# Autodesk Inventor assembly: Base
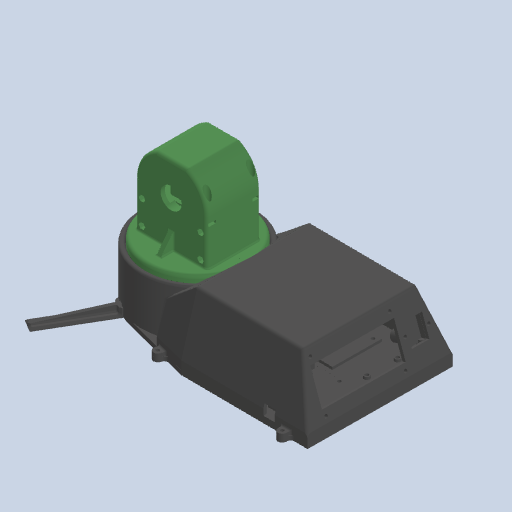
[picture p0: Inventor's stored thumbnail of the model, 512x512]
Saved by Autodesk Inventor 2023 (Build 270158000, 158)
## iProperties
Created: 2024-07-31
Part Number: Base
Document SubType Name: Assembly
Designer: Swoby
Author: Swoby
## Documents named in this file (10)
- C:\Users\Swoby\OneDrive\Plocha\DUM-E\V0.3\NewBase\Base.iam
- C:\Users\Swoby\OneDrive\Plocha\DUM-E\V0.3\NewBase\Base_1L.ipt
- C:\Users\Swoby\OneDrive\Plocha\DUM-E\V0.3\NewBase\Base_1R.ipt
- C:\Users\Swoby\OneDrive\Plocha\DUM-E\V0.3\NewBase\Base_1Up.ipt
- C:\Users\Swoby\OneDrive\Plocha\DUM-E\V0.3\NewBase\Base_2R.ipt
- C:\Users\Swoby\OneDrive\Plocha\DUM-E\V0.3\NewBase\Base_2Leg.ipt
- C:\Users\Swoby\OneDrive\Plocha\DUM-E\V0.3\NewBase\Base_2L.ipt
- C:\Users\Swoby\OneDrive\Plocha\DUM-E\V0.3\NewBase\Clamp_Holder.ipt
- C:\Users\Swoby\OneDrive\Plocha\DUM-E\V0.3\NewBase\Base_Cover.ipt
- C:\Users\Swoby\OneDrive\Plocha\DUM-E\V0.3\NewBase\KeyPad_Holder.ipt
## Components (11 placed, 9 different names)
1. Base_1L:1 — Mate:1, Mate:2, Mate:3, Mate:5, Mate:6, Mate:7, Mate:8
2. Base_1R:1 — Mate:1, Mate:2, Mate:3, Mate:4
3. Base_1Up:1 — Mate:4, Mate:5, Mate:6
4. Base_2R:1 — Mate:7, Mate:8, Mate:11, Mate:12, Mate:13, Flush:3, Mate:16, Mate:17
5. Base_2Leg:1 — Flush:3, Mate:16, Mate:17
6. Base_2L:1 — Mate:11, Mate:12, Mate:13, Mate:14, Flush:2, Mate:15, Mate:18, Mate:19, Mate:20, Mate:21, Mate:22, Mate:23, Flush:4, Flush:5, Mate:24
7. Base_2Leg:2 — Mate:14, Flush:2, Mate:15
8. Clamp_Holder:1 — Mate:18, Mate:19, Mate:22
9. Clamp_Holder:2 — Mate:20, Mate:21, Mate:23
10. Base_Cover:1 — Flush:4, Flush:5, Mate:24, Mate:25, Mate:26, Mate:27
11. KeyPad_Holder:1 — Mate:25, Mate:26, Mate:27
## Relationships (29: Mate 25, Flush 4)
- Mate:1: Base_1L:1 ↔ Base_1R:1
- Mate:2: Base_1L:1 ↔ Base_1R:1
- Mate:3: Base_1L:1 ↔ Base_1R:1
- Mate:4: Base_1R:1 ↔ Base_1Up:1
- Mate:5: Base_1L:1 ↔ Base_1Up:1
- Mate:6: Base_1L:1 ↔ Base_1Up:1
- Mate:7 (0.5 mm): Base_1L:1 ↔ Base_2R:1
- Mate:8: Base_1L:1 ↔ Base_2R:1
- Mate:11: Base_2R:1 ↔ Base_2L:1
- Mate:12: Base_2R:1 ↔ Base_2L:1
- Mate:13: Base_2R:1 ↔ Base_2L:1
- Mate:14: Base_2L:1 ↔ Base_2Leg:2
- Flush:2: Base_2L:1 ↔ Base_2Leg:2
- Mate:15 (0.3 mm): Base_2L:1 ↔ Base_2Leg:2
- Flush:3: Base_2R:1 ↔ Base_2Leg:1
- Mate:16: Base_2R:1 ↔ Base_2Leg:1
- Mate:17 (0.3 mm): Base_2R:1 ↔ Base_2Leg:1
- Mate:18: Base_2L:1 ↔ Clamp_Holder:1
- Mate:19: Base_2L:1 ↔ Clamp_Holder:1
- Mate:20: Base_2L:1 ↔ Clamp_Holder:2
- Mate:21: Base_2L:1 ↔ Clamp_Holder:2
- Mate:22: Base_2L:1 ↔ Clamp_Holder:1
- Mate:23: Base_2L:1 ↔ Clamp_Holder:2
- Flush:4: Base_2L:1 ↔ Base_Cover:1
- Flush:5: Base_2L:1 ↔ Base_Cover:1
- Mate:24: Base_2L:1 ↔ Base_Cover:1
- Mate:25: Base_Cover:1 ↔ KeyPad_Holder:1
- Mate:26: Base_Cover:1 ↔ KeyPad_Holder:1
- Mate:27: Base_Cover:1 ↔ KeyPad_Holder:1
